# Autodesk Inventor assembly: Desk Assembly
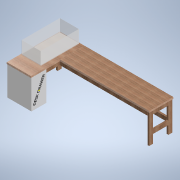
[picture p0: Inventor's stored thumbnail of the model, 180x180]
Saved by Autodesk Inventor 2021 (Build 250183000, 183)
## iProperties
Created: 2019-12-30
Part Number: Desk Assembly
Document SubType Name: Assembly
Designer: Andrew
Author: Andrew
## Documents named in this file (8)
- D:\OneDrive\3D Models\Corner Desk\Desk Assembly.iam
- D:\OneDrive\3D Models\Corner Desk\Desk Top Primary.ipt
- D:\OneDrive\3D Models\Corner Desk\Desk Top Secondary.ipt
- D:\OneDrive\3D Models\Corner Desk\Tank.ipt
- D:\OneDrive\3D Models\Corner Desk\Desk Drawer.ipt
- D:\OneDrive\3D Models\Corner Desk\Frame Secondary.ipt
- D:\OneDrive\3D Models\Corner Desk\Frame Primary.ipt
- D:\OneDrive\3D Models\Corner Desk\Frame Single.ipt
## Components (7 placed, 7 different names)
1. Desk Top Primary:1 — Flush:1, Flush:2, Flush:3
2. Desk Top Secondary:1 — Flush:4, Flush:5, Flush:6, Mate:1, Flush:7, Flush:8, Mate:2, Flush:9, Flush:10
3. Tank:1 — Mate:1, Flush:7, Flush:8
4. Desk Drawer:1 — Mate:2, Flush:9, Flush:10
5. Frame Secondary:1 — Flush:11, Flush:12, Flush:13
6. Frame Primary:1 — Flush:14, Flush:15, Flush:16
7. Frame Single:1 — Flush:17, Flush:18, Flush:19
## Relationships (21: Flush 19, Mate 2)
- Flush:1: Desk Top Primary:1
- Flush:2: Desk Top Primary:1
- Flush:3: Desk Top Primary:1
- Flush:4: Desk Top Secondary:1
- Flush:5: Desk Top Secondary:1
- Flush:6: Desk Top Secondary:1
- Mate:1: Desk Top Secondary:1 ↔ Tank:1
- Flush:7 (25.4 mm): Desk Top Secondary:1 ↔ Tank:1
- Flush:8 (25.4 mm): Desk Top Secondary:1 ↔ Tank:1
- Mate:2: Desk Top Secondary:1 ↔ Desk Drawer:1
- Flush:9: Desk Top Secondary:1 ↔ Desk Drawer:1
- Flush:10 (-12.7 mm): Desk Top Secondary:1 ↔ Desk Drawer:1
- Flush:11: Frame Secondary:1
- Flush:12: Frame Secondary:1
- Flush:13: Frame Secondary:1
- Flush:14: Frame Primary:1
- Flush:15: Frame Primary:1
- Flush:16: Frame Primary:1
- Flush:17: Frame Single:1
- Flush:18: Frame Single:1
- Flush:19: Frame Single:1
